# Autodesk Inventor assembly: Pull Tester
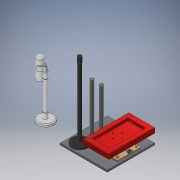
[picture p0: Inventor's stored thumbnail of the model, 180x180]
Saved by Autodesk Inventor 2019.4 (Build 234330000, 330)
## iProperties
Created: 2020-11-12
Part Number: Pull Tester
Document SubType Name: Assembly
Designer: caleb
Author: caleb
## Documents named in this file (10)
- C:\Users\cfang\Desktop\nebraska-silicon-lab\CAD\Pull Tester\Pull Tester.iam
- C:\Users\cfang\Desktop\nebraska-silicon-lab\CAD\Pull Tester\Chuck.ipt
- C:\Users\cfang\Desktop\nebraska-silicon-lab\CAD\Pull Tester\step_12692.ipt
- C:\Users\cfang\Desktop\nebraska-silicon-lab\CAD\Pull Tester\90128A211_ZNC-PLTD ALLOY STL SCKT HEAD CAP SCREW.ipt
- C:\Users\cfang\Desktop\nebraska-silicon-lab\CAD\Pull Tester\step_12694.ipt
- C:\Users\cfang\Desktop\nebraska-silicon-lab\CAD\Pull Tester\FTK100.ipt
- C:\Users\cfang\Desktop\nebraska-silicon-lab\CAD\Pull Tester\92421A642_BRASS FLARED-COLLAR KNURLED-HEAD THUMB SCREWS.ipt
- C:\Users\cfang\Desktop\nebraska-silicon-lab\CAD\Pull Tester\49985A250_ANY-WHICH-WAY POSITIONING ARM.ipt
- C:\Users\cfang\Desktop\nebraska-silicon-lab\CAD\Pull Tester\49985A240_ANY-WHICH-WAY POSITIONING ARM.ipt
- C:\Users\cfang\Desktop\nebraska-silicon-lab\CAD\Pull Tester\Camera with Clip.iam
## Components (14 placed, 9 different names)
1. Chuck:1 — Insert:22, Insert:23, Insert:24, Angle:4, Insert:26, Angle:6
2. step_12692:1 — Mate:3, Angle:5, Insert:25, Insert:26
3. 90128A211_ZNC-PLTD ALLOY STL SCKT HEAD CAP SCREW:1 — Insert:24
4. 90128A211_ZNC-PLTD ALLOY STL SCKT HEAD CAP SCREW:2 — Insert:23
5. 90128A211_ZNC-PLTD ALLOY STL SCKT HEAD CAP SCREW:3 — Insert:22
6. step_12694:1 — Mate:2, Angle:2, Flush:1, Flush:2, Mate:3, Insert:25, Insert:27, Insert:28, Insert:29, Insert:30
7. FTK100:1 — Mate:2, Angle:2, Flush:1, Flush:2, Angle:4, Angle:5, Angle:6, Mate:4, Mate:5
8. 92421A642_BRASS FLARED-COLLAR KNURLED-HEAD THUMB SCREWS:1 — Insert:29
9. 92421A642_BRASS FLARED-COLLAR KNURLED-HEAD THUMB SCREWS:2 — Insert:27
10. 92421A642_BRASS FLARED-COLLAR KNURLED-HEAD THUMB SCREWS:3 — Insert:30
11. 92421A642_BRASS FLARED-COLLAR KNURLED-HEAD THUMB SCREWS:4 — Insert:28
12. 49985A250_ANY-WHICH-WAY POSITIONING ARM:1 — Mate:4
13. 49985A240_ANY-WHICH-WAY POSITIONING ARM:1 — Mate:5, Insert:31
14. Camera with Clip:1 [sub-assembly] — Insert:31
## Relationships (20: Insert 10, Mate 4, Angle 4, Flush 2)
- Insert:22: Chuck:1 ↔ 90128A211_ZNC-PLTD ALLOY STL SCKT HEAD CAP SCREW:3
- Insert:23: Chuck:1 ↔ 90128A211_ZNC-PLTD ALLOY STL SCKT HEAD CAP SCREW:2
- Insert:24: Chuck:1 ↔ 90128A211_ZNC-PLTD ALLOY STL SCKT HEAD CAP SCREW:1
- Mate:2: step_12694:1 ↔ FTK100:1
- Angle:2 (0 deg): step_12694:1 ↔ FTK100:1
- Flush:1 (-10.16 mm): step_12694:1 ↔ FTK100:1
- Flush:2 (64.77 mm): step_12694:1 ↔ FTK100:1
- Angle:4 (0 deg): Chuck:1 ↔ FTK100:1
- Mate:3: step_12692:1 ↔ step_12694:1
- Angle:5 (0 deg): step_12692:1 ↔ FTK100:1
- Insert:25: step_12692:1 ↔ step_12694:1
- Insert:26: Chuck:1 ↔ step_12692:1
- Angle:6 (0 deg): Chuck:1 ↔ FTK100:1
- Insert:27: step_12694:1 ↔ 92421A642_BRASS FLARED-COLLAR KNURLED-HEAD THUMB SCREWS:2
- Insert:28: step_12694:1 ↔ 92421A642_BRASS FLARED-COLLAR KNURLED-HEAD THUMB SCREWS:4
- Insert:29: step_12694:1 ↔ 92421A642_BRASS FLARED-COLLAR KNURLED-HEAD THUMB SCREWS:1
- Insert:30: step_12694:1 ↔ 92421A642_BRASS FLARED-COLLAR KNURLED-HEAD THUMB SCREWS:3
- Mate:4: FTK100:1 ↔ 49985A250_ANY-WHICH-WAY POSITIONING ARM:1
- Mate:5: FTK100:1 ↔ 49985A240_ANY-WHICH-WAY POSITIONING ARM:1
- Insert:31: 49985A240_ANY-WHICH-WAY POSITIONING ARM:1 ↔ Camera with Clip:1
